# Autodesk Inventor assembly: ChestController
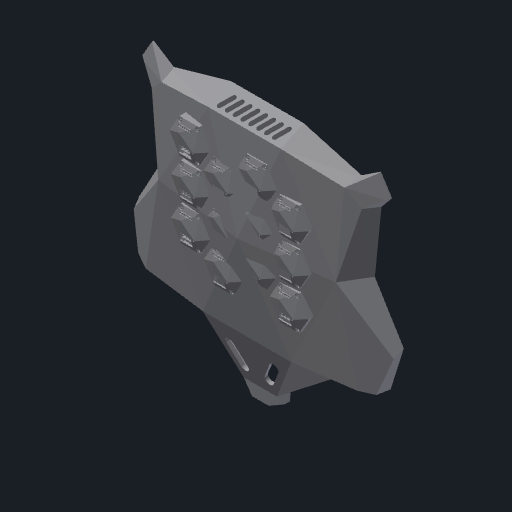
[picture p0: Inventor's stored thumbnail of the model, 512x512]
Saved by Autodesk Inventor 2025.2 (Build 292293000, 293)
## iProperties
Created: 2025-10-06
Part Number: ChestController
Document SubType Name: Assembly
Designer: valer
Author: valer
## Documents named in this file (3)
- C:\Users\valer\Desktop\str1ker\cad\ChestController.iam
- C:\Users\valer\Desktop\str1ker\cad\ControlBoard.ipt
- C:\Users\valer\Desktop\str1ker\cad\ArmDriver.iam
## Components (13 placed, 2 different names)
1. ControlBoard:1 — Flush:1, Flush:2, Flush:3, Mate:1
2. ArmDriver:1 [sub-assembly] — Angle:1, Mate:1
3. ArmDriver:2 [sub-assembly]
4. ArmDriver:3 [sub-assembly]
5. ArmDriver:4 [sub-assembly]
6. ArmDriver:5 [sub-assembly]
7. ArmDriver:6 [sub-assembly]
8. ArmDriver:7 [sub-assembly]
9. ArmDriver:8 [sub-assembly]
10. ArmDriver:9 [sub-assembly]
11. ArmDriver:10 [sub-assembly]
12. ArmDriver:11 [sub-assembly]
13. ArmDriver:12 [sub-assembly]
## Relationships (5: Flush 3, Angle 1, Mate 1)
- Flush:1: ControlBoard:1
- Flush:2: ControlBoard:1
- Flush:3: ControlBoard:1
- Angle:1 (180 deg): ArmDriver:1
- Mate:1: ControlBoard:1 ↔ ArmDriver:1
